# Autodesk Inventor assembly: M2 Hex Nuts
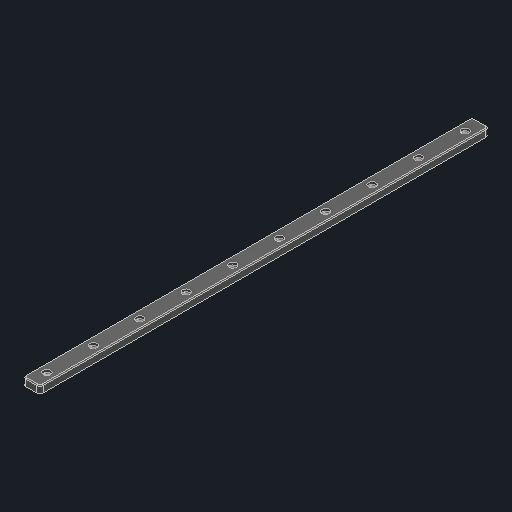
[picture p0: Inventor's stored thumbnail of the model, 512x512]
Saved by Autodesk Inventor 2025.1 (Build 291241020, 241B)
## iProperties
Created: 2025-05-11
Part Number: M2 Hex Nuts
Document SubType Name: Assembly
Designer: Joshua Eah
Author: Joshua Eah
## Documents named in this file (3)
- C:\Users\Joshua Eah\Documents\Voron 0.2\CAD\Master Assembly\M2 Hex Nuts.iam
- C:\Users\Joshua Eah\Documents\Voron 0.2\CAD\Master Assembly\M2 Hex Adapter.ipt
- C:\Users\Joshua Eah\Documents\Voron 0.2\CAD\Master Assembly\Hardware\M2 Hex Nut.ipt
## Components (11 placed, 2 different names)
1. M2 Hex Adapter:1 — Insert:1, Insert:2, Insert:3, Insert:4, Insert:5, Insert:6, Insert:7, Insert:8, Insert:9, Insert:10
2. M2 Hex Nut:1 — Insert:9
3. M2 Hex Nut:2 — Insert:7
4. M2 Hex Nut:3 — Insert:10
5. M2 Hex Nut:4 — Insert:2
6. M2 Hex Nut:5 — Insert:5
7. M2 Hex Nut:6 — Insert:1
8. M2 Hex Nut:7 — Insert:3
9. M2 Hex Nut:8 — Insert:8
10. M2 Hex Nut:9 — Insert:6
11. M2 Hex Nut:10 — Insert:4
## Relationships (10: Insert 10)
- Insert:1: M2 Hex Adapter:1 ↔ M2 Hex Nut:6
- Insert:2: M2 Hex Adapter:1 ↔ M2 Hex Nut:4
- Insert:3: M2 Hex Adapter:1 ↔ M2 Hex Nut:7
- Insert:4: M2 Hex Adapter:1 ↔ M2 Hex Nut:10
- Insert:5: M2 Hex Adapter:1 ↔ M2 Hex Nut:5
- Insert:6: M2 Hex Adapter:1 ↔ M2 Hex Nut:9
- Insert:7: M2 Hex Adapter:1 ↔ M2 Hex Nut:2
- Insert:8: M2 Hex Adapter:1 ↔ M2 Hex Nut:8
- Insert:9: M2 Hex Adapter:1 ↔ M2 Hex Nut:1
- Insert:10: M2 Hex Adapter:1 ↔ M2 Hex Nut:3
